# Autodesk Inventor assembly: gps mount assembly
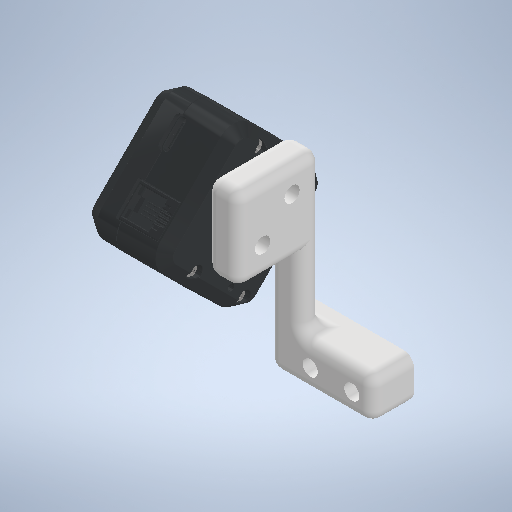
[picture p0: Inventor's stored thumbnail of the model, 512x512]
Saved by Autodesk Inventor 2025.1 (Build 291241020, 241B)
## iProperties
Created: 2025-01-10
Part Number: gps mount assembly
Document SubType Name: Assembly
Designer: AtuStem
Author: AtuStem
## Documents named in this file (3)
- C:\Users\AtuStem\Documents\GitHub\ATUM-V5RC-High-Stakes-CAD\Additional Parts\gps mount assembly.iam
- C:\Users\AtuStem\Documents\GitHub\ATUM-V5RC-High-Stakes-CAD\Additional Parts\real deal gps holder.ipt
- C:\Users\AtuStem\Documents\GitHub\ATUM-V5RC-High-Stakes-CAD\VEX-CAD-Inventor\Electronics\Sensors\V5 GPS Sensor.ipt
## Components (2 placed, 2 different names)
1. real deal gps holder:1 — Mate:1, Mate:2, Mate:3
2. V5 GPS Sensor:1 — Mate:1, Mate:2, Mate:3
## Relationships (3: Mate 3)
- Mate:1: real deal gps holder:1 ↔ V5 GPS Sensor:1
- Mate:2: real deal gps holder:1 ↔ V5 GPS Sensor:1
- Mate:3: real deal gps holder:1 ↔ V5 GPS Sensor:1
